# Autodesk Inventor assembly: EngravingJigAssemblyBack
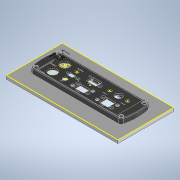
[picture p0: Inventor's stored thumbnail of the model, 180x180]
Saved by Autodesk Inventor 2021 (Build 250183000, 183)
## iProperties
Created: 2021-02-01
Part Number: EngravingJigAssemblyBack
Document SubType Name: Assembly
Designer: Viktor
Author: Viktor
## Documents named in this file (3)
- C:\Users\Viktor\Google Drive\Unicorn 2020\CAD_V2\Manufacturing\EngravingJigAssemblyBack.iam
- C:\Users\Viktor\Google Drive\Unicorn 2020\CAD_V2\Manufacturing\EngravingJig.ipt
- C:\Users\Viktor\Google Drive\Unicorn 2020\CAD_V2\Back_Panel\Panel\1009799_3D_Back.ipt
## Components (2 placed, 2 different names)
1. EngravingJig:1 — Mate:1, Mate:2, Mate:3
2. 1009799_3D_Back:1 — Mate:1, Mate:2, Mate:3
## Relationships (3: Mate 3)
- Mate:1: EngravingJig:1 ↔ 1009799_3D_Back:1
- Mate:2: EngravingJig:1 ↔ 1009799_3D_Back:1
- Mate:3: EngravingJig:1 ↔ 1009799_3D_Back:1
